# Autodesk Inventor assembly: housingLibAssembly
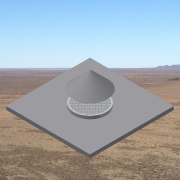
[picture p0: Inventor's stored thumbnail of the model, 180x180]
Saved by Autodesk Inventor 2014 SP1 (Build 180222100, 222)
## iProperties
Created: 2014-05-23
Part Number: housingLibAssembly
Document SubType Name: Assembly
Designer: Dave
Author: Dave
## Documents named in this file (4)
- C:\Users\Dave\Desktop\hera-cad\Node\housingLibAssembly.iam
- C:\Users\Dave\Desktop\hera-cad\Node\housingLid.ipt
- C:\Users\Dave\Desktop\hera-cad\Node\lidHoneycomb.ipt
- C:\Users\Dave\Desktop\hera-cad\Node\chimneyCap.ipt
## Components (3 placed, 3 different names)
1. housingLid:1 — Insert:1
2. lidHoneycomb:1 — Insert:1, Insert:2
3. chimneyCap:1 — Insert:2
## Relationships (2: Insert 2)
- Insert:1: housingLid:1 ↔ lidHoneycomb:1
- Insert:2 (-101.6 mm): lidHoneycomb:1 ↔ chimneyCap:1
